# Autodesk Inventor assembly: K1S4andMirror
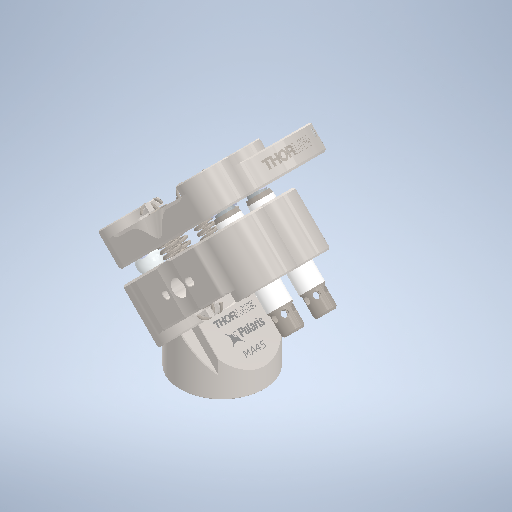
[picture p0: Inventor's stored thumbnail of the model, 512x512]
Saved by Autodesk Inventor 2025.2 (Build 292293000, 293)
## iProperties
Created: 2023-10-20
Part Number: K1S4andMirror
Document SubType Name: Assembly
Designer: S227943
Author: S227943
## Documents named in this file (4)
- C:\Users\monolithic\Documents\GitHub\CAD\Monolith\John\2026_2_9_CondensedCTASLMBaseplate\Assembly\Components\K1S4andMirrorNoPost.iam
- C:\Users\monolithic\Documents\GitHub\CAD\Monolith\John\Altair_PowellBaseplate_SPIM_ASLM_CTASLM\Assembly\SubAssemblies\POLARIS-K1S4.ipt
- C:\Users\monolithic\Documents\GitHub\CAD\Monolith\John\Altair_PowellBaseplate_SPIM_ASLM_CTASLM\Assembly\SubAssemblies\POLARIS-MA45.ipt
- C:\Users\monolithic\Documents\GitHub\CAD\Monolith\John\Altair_PowellBaseplate_SPIM_ASLM_CTASLM\Assembly\SubAssemblies\PF10-03-P01.ipt
## Components (3 placed, 3 different names)
1. POLARIS-K1S4:1 — Mate:1, Mate:2, Angle:1, Mate:3, Mate:4
2. POLARIS-MA45:1 — Mate:1, Mate:2, Angle:1
3. PF10-03-P01:1 — Mate:3, Mate:4
## Relationships (5: Mate 4, Angle 1)
- Mate:1: POLARIS-K1S4:1 ↔ POLARIS-MA45:1
- Mate:2: POLARIS-K1S4:1 ↔ POLARIS-MA45:1
- Angle:1 (90 deg): POLARIS-K1S4:1 ↔ POLARIS-MA45:1
- Mate:3: POLARIS-K1S4:1 ↔ PF10-03-P01:1
- Mate:4: POLARIS-K1S4:1 ↔ PF10-03-P01:1
